# Autodesk Inventor assembly: arm stack
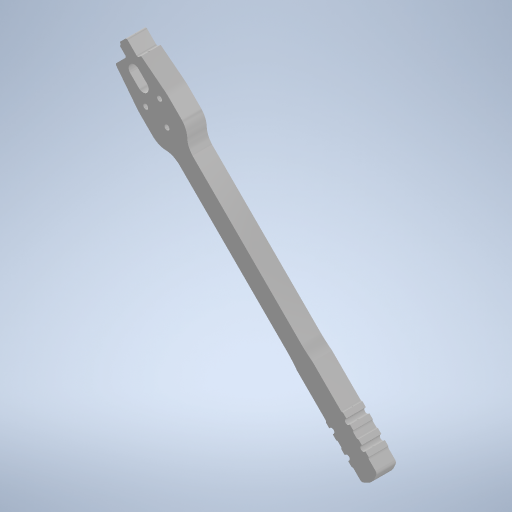
[picture p0: Inventor's stored thumbnail of the model, 512x512]
Saved by Autodesk Inventor 2023 (Build 270158000, 158)
## iProperties
Created: 2023-01-22
Part Number: arm stack
Document SubType Name: Assembly
Designer: Steven
Author: Steven
## Documents named in this file (2)
- Y:\FPV drone stuff\0 Street League\Frames\experimental-quad-frames\Nightstick MAX\arm stack.iam
- Y:\FPV drone stuff\0 Street League\Frames\experimental-quad-frames\Nightstick MAX\arm NightStickmax.ipt
## Components (2 placed, 1 different names)
1. arm NightStickmax:1 — Mate:1, Mate:2, Mate:3
2. arm NightStickmax:2 — Mate:1, Flush:1, Flush:2, Flush:3, Mate:2, Mate:3
## Relationships (6: Mate 3, Flush 3)
- Mate:1: arm NightStickmax:1 ↔ arm NightStickmax:2
- Flush:1: arm NightStickmax:2
- Flush:2: arm NightStickmax:2
- Flush:3: arm NightStickmax:2
- Mate:2: arm NightStickmax:1 ↔ arm NightStickmax:2
- Mate:3: arm NightStickmax:1 ↔ arm NightStickmax:2
